# Autodesk Inventor assembly: MIR_HbSocketU02ForChild
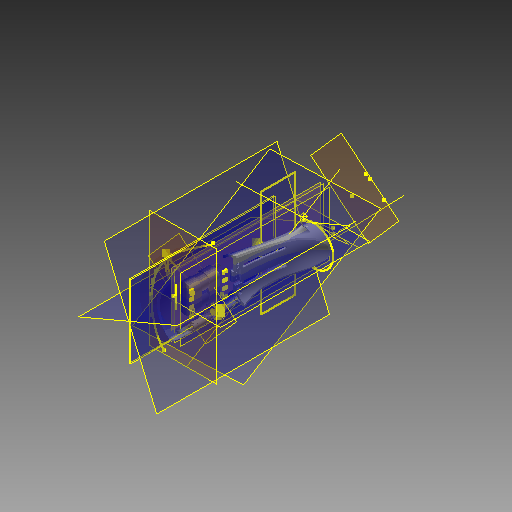
[picture p0: Inventor's stored thumbnail of the model, 512x512]
Saved by Autodesk Inventor 2018.1 (Build 221171000, 171)
## iProperties
Created: 2015-02-09
Part Number: MIR_HbSocketU02ForChild
Document SubType Name: Assembly
Designer: sktom
Author: Yamaura
## Documents named in this file (10)
- D:\CloudStrage\OneDrive\CAD\MAJ\hackberry\HACKberry-hardware\3D_69%inlength\Inventor\HbSocketU02ForChild\MIR_HbSocketU02ForChild.iam
- D:\CloudStrage\OneDrive\CAD\MAJ\hackberry\HACKberry-hardware\3D_69%inlength\Inventor\HbSocketU02ForChild\MIR_HbBatteryDoorKnob03.ipt
- D:\CloudStrage\OneDrive\CAD\MAJ\hackberry\HACKberry-hardware\3D_69%inlength\Inventor\HbSocketU02ForChild\MIR_HbBatteryHingeC03.ipt
- D:\CloudStrage\OneDrive\CAD\MAJ\hackberry\HACKberry-hardware\3D_69%inlength\Inventor\HbSocketU02ForChild\MIR_HbBatteryHingeB03.ipt
- D:\CloudStrage\OneDrive\CAD\MAJ\hackberry\HACKberry-hardware\3D_69%inlength\Inventor\HbSocketU02ForChild\MIR_HbBatteryHingeA03.ipt
- D:\CloudStrage\OneDrive\CAD\MAJ\hackberry\HACKberry-hardware\3D_69%inlength\Inventor\HbSocketU02ForChild\MIR_HbBatteryDoor03.ipt
- D:\CloudStrage\OneDrive\CAD\MAJ\hackberry\HACKberry-hardware\3D_69%inlength\Inventor\HbSocketU02ForChild\MIR_HbMainFrameA01.ipt
- D:\CloudStrage\OneDrive\CAD\MAJ\hackberry\HACKberry-hardware\3D_69%inlength\Inventor\HbSocketU02ForChild\MIR_HbMainFrameB01.ipt
- D:\CloudStrage\OneDrive\CAD\MAJ\hackberry\HACKberry-hardware\3D_69%inlength\Inventor\HbSocketU02ForChild\MIR_HbBatteryDoorLever03.ipt
- D:\CloudStrage\OneDrive\CAD\MAJ\hackberry\HACKberry-hardware\3D_69%inlength\Inventor\HbBatteryCase\MIR_HbBatteryCase.iam
## Components (12 placed, 9 different names)
1. MIR_HbBatteryHingeC03:1 — 挿入:7, 挿入:6
2. MIR_HbBatteryHingeB03:1 — 挿入:9, 挿入:8
3. MIR_HbBatteryHingeA03:1 — 挿入:11, 挿入:10
4. MIR_HbBatteryDoor03:1 — 挿入:11, 挿入:10, 挿入:9, 挿入:8, 挿入:7, 挿入:6, 挿入:12
5. MIR_HbMainFrameA01:1 — 挿入:5, 挿入:4, メイト:2, メイト:1
6. MIR_HbBatteryDoorKnob03:2 — メイト:2, メイト:1, 挿入:3
7. MIR_HbMainFrameB01:1 — 挿入:12, 挿入:5, 挿入:4, メイト:4
8. MIR_HbBatteryCase:1 [sub-assembly] — メイト:4
9. MIR_HbBatteryDoorKnob03:1
10. MIR_HbBatteryDoorKnob03:3
11. MIR_HbBatteryDoorLever03:1
12. MIR_HbBatteryDoorLever03:2 — 挿入:3
## Component patterns: (2 elements, first: MIR_HbBatteryDoorKnob03:1), (2 elements, first: MIR_HbBatteryDoorLever03:1)
## Relationships (13: Insert 10, Mate 3)
- 挿入:11 [Insert]: MIR_HbBatteryHingeA03:1 ↔ MIR_HbBatteryDoor03:1
- 挿入:10 [Insert]: MIR_HbBatteryHingeA03:1 ↔ MIR_HbBatteryDoor03:1
- 挿入:9 [Insert]: MIR_HbBatteryHingeB03:1 ↔ MIR_HbBatteryDoor03:1
- 挿入:8 [Insert]: MIR_HbBatteryHingeB03:1 ↔ MIR_HbBatteryDoor03:1
- 挿入:7 [Insert]: MIR_HbBatteryHingeC03:1 ↔ MIR_HbBatteryDoor03:1
- 挿入:6 [Insert]: MIR_HbBatteryHingeC03:1 ↔ MIR_HbBatteryDoor03:1
- 挿入:12 [Insert]: MIR_HbBatteryDoor03:1 ↔ MIR_HbMainFrameB01:1
- 挿入:5 [Insert]: MIR_HbMainFrameA01:1 ↔ MIR_HbMainFrameB01:1
- 挿入:4 [Insert]: MIR_HbMainFrameA01:1 ↔ MIR_HbMainFrameB01:1
- メイト:2 [Mate]: MIR_HbMainFrameA01:1 ↔ MIR_HbBatteryDoorKnob03:2
- メイト:1 [Mate]: MIR_HbMainFrameA01:1 ↔ MIR_HbBatteryDoorKnob03:2
- メイト:4 [Mate]: MIR_HbMainFrameB01:1 ↔ MIR_HbBatteryCase:1
- 挿入:3 [Insert]: MIR_HbBatteryDoorKnob03:2 ↔ MIR_HbBatteryDoorLever03:2
